# Autodesk Inventor assembly: mg996r_base_motor_with_axis
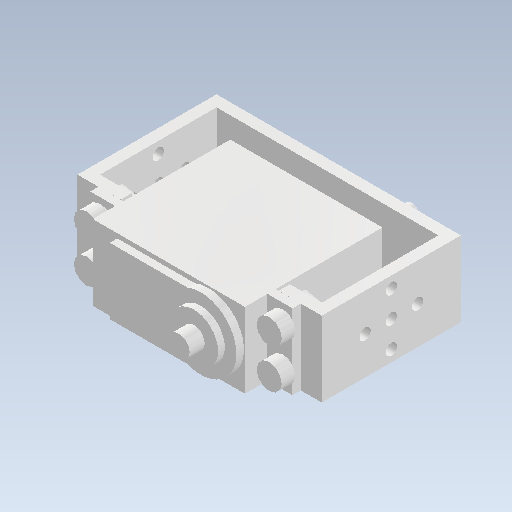
[picture p0: Inventor's stored thumbnail of the model, 512x512]
Saved by Autodesk Inventor 2021.4 (Build 254397000, 397)
## iProperties
Created: 2022-07-26
Part Number: mg996r_base_motor_with_axis
Document SubType Name: Assembly
Designer: isamu
Author: isamu
## Documents named in this file (3)
- D:\personal_projects\robot\inventor\2021_matlab_compat _v2\motor_with_frames\mg996r_base_motor_with_axis.iam
- D:\personal_projects\robot\inventor\2021_matlab_compat _v2\motor\mg996r_motor_with_screws.iam
- D:\personal_projects\robot\inventor\2021_matlab_compat _v2\servo_frames\servo_frame_with_nuts.iam
## Components (2 placed, 2 different names)
1. mg996r_motor_with_screws:1 [sub-assembly] — Mate:1, Mate:2, Mate:3
2. servo_frame_with_nuts:1 [sub-assembly] — Mate:1, Mate:2, Mate:3
## Relationships (3: Mate 3)
- Mate:1: mg996r_motor_with_screws:1 ↔ servo_frame_with_nuts:1
- Mate:2: mg996r_motor_with_screws:1 ↔ servo_frame_with_nuts:1
- Mate:3: mg996r_motor_with_screws:1 ↔ servo_frame_with_nuts:1
